# Autodesk Inventor assembly: mould assembly
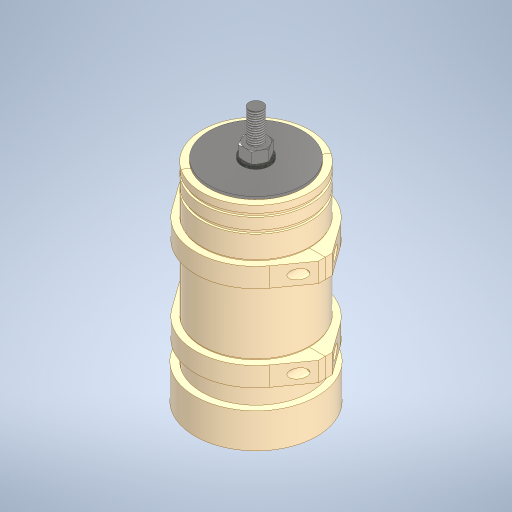
[picture p0: Inventor's stored thumbnail of the model, 512x512]
Saved by Autodesk Inventor 2024 (Build 280153020, 153B)
## iProperties
Created: 2023-06-12
Part Number: mould assembly
Document SubType Name: Assembly
Designer: OKESH
Author: OKESH
## Documents named in this file (10)
- C:\Users\OKESH\Documents\mould assembly.iam
- C:\Users\OKESH\Documents\half cylinder.ipt
- C:\Users\OKESH\Documents\clamp.ipt
- C:\Users\OKESH\Documents\bottom.ipt
- C:\Users\OKESH\Documents\center.ipt
- C:\Users\OKESH\Documents\top.ipt
- C:\Users\OKESH\Documents\Inventor\Content Center Files\R2024\en-US\ISO 7091\ISO 7091 - ST 10 - 100 HV.ipt
- C:\Users\OKESH\Documents\Inventor\Content Center Files\R2024\en-US\ANSI B 18.2.4.1 M(1)\ANSI B 18.2.4.1 M - M10 x 1.5Style 1.ipt
- C:\Users\OKESH\Documents\Inventor\Content Center Files\R2024\en-US\AS 1110\AS 1110 - M5 x 10.ipt
- C:\Users\OKESH\Documents\seal.ipt
## Components (14 placed, 9 different names)
1. half cylinder:1 — Flush:1, Mate:1, Mate:8, Mate:9, Mate:10, Mate:11, Mate:19
2. half cylinder:2 — Flush:1, Mate:1, Mate:19
3. clamp:1 — Mate:2, Mate:3, Mate:4, Mate:8
4. clamp:2 — Mate:5, Mate:6, Mate:7, Mate:9
5. clamp:3 — Mate:5, Mate:6, Mate:7
6. clamp:4 — Mate:2, Mate:3, Mate:4
7. bottom:1 — Mate:10, Mate:11, Mate:12, Mate:13, Insert:1
8. center:1 — Mate:12, Mate:13, Mate:14, Mate:15, Mate:17, Mate:20, Mate:21
9. top:1 — Mate:14, Mate:16
10. ISO 7091 ST 10 - 100 HV:1 — Mate:15, Mate:16, Mate:18
11. Hex Nut Metric M10 x 1.5:1 — Mate:17, Mate:18
12. AS 1110 - Metric M5 x 10:1 — Insert:1
13. seal:1 — Mate:20
14. seal:2 — Mate:21
## Relationships (23: Mate 21, Flush 1, Insert 1)
- Flush:1: half cylinder:1 ↔ half cylinder:2
- Mate:1: half cylinder:1 ↔ half cylinder:2
- Mate:2: clamp:1 ↔ clamp:4
- Mate:3: clamp:1 ↔ clamp:4
- Mate:4: clamp:1 ↔ clamp:4
- Mate:5: clamp:2 ↔ clamp:3
- Mate:6: clamp:2 ↔ clamp:3
- Mate:7: clamp:2 ↔ clamp:3
- Mate:8: half cylinder:1 ↔ clamp:1
- Mate:9: half cylinder:1 ↔ clamp:2
- Mate:10: half cylinder:1 ↔ bottom:1
- Mate:11: half cylinder:1 ↔ bottom:1
- Mate:12: bottom:1 ↔ center:1
- Mate:13: bottom:1 ↔ center:1
- Mate:14: center:1 ↔ top:1
- Mate:15: center:1 ↔ ISO 7091 ST 10 - 100 HV:1
- Mate:16: top:1 ↔ ISO 7091 ST 10 - 100 HV:1
- Mate:17: center:1 ↔ Hex Nut Metric M10 x 1.5:1
- Mate:18: ISO 7091 ST 10 - 100 HV:1 ↔ Hex Nut Metric M10 x 1.5:1
- Insert:1: bottom:1 ↔ AS 1110 - Metric M5 x 10:1
- Mate:19: half cylinder:1 ↔ half cylinder:2
- Mate:20: center:1 ↔ seal:1
- Mate:21: center:1 ↔ seal:2
